# Autodesk Inventor assembly: ESTOP Complete Assembley
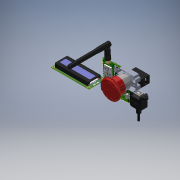
[picture p0: Inventor's stored thumbnail of the model, 180x180]
Saved by Autodesk Inventor 2019 (Build 230136000, 136)
## iProperties
Created: 2019-10-09
Part Number: ESTOP Complete Assembley
Document SubType Name: Assembly
Designer: rybit
Author: rybit
## Documents named in this file (6)
- I:\CMR4GR\Documents\Inventor\ESTOP V2\ESTOP Complete Assembley.iam
- I:\CMR4GR\Documents\Inventor\ESTOP V2\ESTOP V2 PCB.iam
- I:\CMR4GR\Documents\Inventor\ESTOP V2\LCD.iam
- I:\CMR4GR\Documents\Inventor\ESTOP V2\Mushroom Switch.ipt
- I:\CMR4GR\Documents\Inventor\ESTOP V2\USB Cable B Male to B Female 90 degrees_Assembly.iam
- I:\CMR4GR\Documents\Inventor\ESTOP V2\Antenna_D‚faut.iam
## Components (5 placed, 5 different names)
1. ESTOP V2 PCB:1 [sub-assembly] — Insert:1
2. LCD:1 [sub-assembly]
3. Mushroom Switch:1
4. USB Cable B Male to B Female 90 degrees_Assembly:1 [sub-assembly]
5. Antenna_D‚faut:1 [sub-assembly] — Insert:1
## Relationships (1: Insert 1)
- Insert:1 (-3.5052 mm): ESTOP V2 PCB:1 ↔ Antenna_D‚faut:1
